# Autodesk Inventor assembly: SHOCK ABSORBER
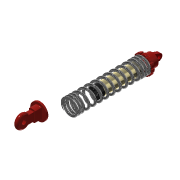
[picture p0: Inventor's stored thumbnail of the model, 180x180]
Saved by Autodesk Inventor 2019 (Build 230136000, 136)
## iProperties
Created: 2023-06-17
Part Number: SHOCK ABSORBER
Document SubType Name: Assembly
Designer: Fransic
Author: Fransic
## Documents named in this file (8)
- C:\Users\Fransic\Documents\Inventor\Shock Absorber\SHOCK ABSORBER.iam
- C:\Users\Fransic\Documents\Inventor\Shock Absorber\TOP STRUT MOUNT.ipt
- C:\Users\Fransic\Documents\Inventor\Shock Absorber\ADJUSTABLE DISC.ipt
- C:\Users\Fransic\Documents\Inventor\Shock Absorber\SPRING.ipt
- C:\Users\Fransic\Documents\Inventor\Shock Absorber\OIL RING.ipt
- C:\Users\Fransic\Documents\Inventor\Shock Absorber\BASE VALVE.ipt
- C:\Users\Fransic\Documents\Inventor\Shock Absorber\PISTON GUIDE.ipt
- C:\Users\Fransic\Documents\Inventor\Shock Absorber\STRUT MOUNT.ipt
## Components (7 placed, 7 different names)
1. ADJUSTABLE DISC:1 — Mate:1, Mate:2
2. SPRING:1 — Mate:3
3. TOP STRUT MOUNT:1 — Mate:1, Mate:2, Mate:3, Mate:5, Mate:6, Mate:7, Mate:9, Mate:10
4. OIL RING:1 — Mate:5, Mate:8
5. BASE VALVE:2 — Mate:6, Mate:7, Mate:8
6. PISTON GUIDE:1 — Mate:9, Mate:10
7. STRUT MOUNT:2
## Relationships (9: Mate 9)
- Mate:1: ADJUSTABLE DISC:1 ↔ TOP STRUT MOUNT:1
- Mate:2: ADJUSTABLE DISC:1 ↔ TOP STRUT MOUNT:1
- Mate:3: SPRING:1 ↔ TOP STRUT MOUNT:1
- Mate:5: TOP STRUT MOUNT:1 ↔ OIL RING:1
- Mate:6: TOP STRUT MOUNT:1 ↔ BASE VALVE:2
- Mate:7 (30 mm): TOP STRUT MOUNT:1 ↔ BASE VALVE:2
- Mate:8: OIL RING:1 ↔ BASE VALVE:2
- Mate:9: TOP STRUT MOUNT:1 ↔ PISTON GUIDE:1
- Mate:10: TOP STRUT MOUNT:1 ↔ PISTON GUIDE:1
